# Autodesk Inventor assembly: DriverStation-ver3-1111-2021
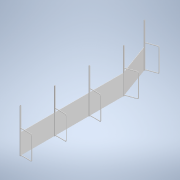
[picture p0: Inventor's stored thumbnail of the model, 180x180]
Saved by Autodesk Inventor 2021 (Build 250183000, 183)
## iProperties
Created: 2021-03-02
Part Number: DriverStation-ver3-1111-2021
Document SubType Name: Assembly
Designer: CMurray
Author: CMurray
## Documents named in this file (3)
- F:\PHRC CADD 2021\2021 Game Design Challenge\Player Station\Assemblies\DriverStation-ver3-1111-2021.iam
- F:\PHRC CADD 2021\2021 Game Design Challenge\Player Station\Parts\StationBase-ver1-1111-2021.ipt
- F:\PHRC CADD 2021\2021 Game Design Challenge\Player Station\Parts\StationDivider-ver1-1111-2021.iam
## Components (9 placed, 2 different names)
1. StationBase-ver1-1111-2021:1 — Mate:1, Flush:1, Flush:2, Flush:3, Mate:2, Flush:4, Flush:7, Flush:8, Flush:11, Flush:12
2. StationDivider-ver1-1111-2021:1 [sub-assembly] — Mate:1, Flush:1, Flush:2, Mate:6
3. StationDivider-ver1-1111-2021:2 [sub-assembly] — Flush:3, Mate:2, Flush:4, Mate:4
4. StationBase-ver1-1111-2021:2 — Mate:4, Flush:7, Flush:8, Flush:13, Mate:9, Flush:16, Angle:1
5. StationBase-ver1-1111-2021:3 — Flush:11, Flush:12, Mate:6
6. StationDivider-ver1-1111-2021:4 [sub-assembly]
7. StationBase-ver1-1111-2021:4 — Flush:13, Mate:8, Flush:14, Flush:15, Mate:10, Angle:1
8. StationDivider-ver1-1111-2021:5 [sub-assembly] — Mate:8, Flush:14, Flush:15, Angle:2
9. StationDivider-ver1-1111-2021:6 [sub-assembly] — Mate:9, Flush:16, Mate:10, Angle:2
## Relationships (24: Flush 14, Mate 8, Angle 2)
- Mate:1: StationBase-ver1-1111-2021:1 ↔ StationDivider-ver1-1111-2021:1
- Flush:1: StationBase-ver1-1111-2021:1 ↔ StationDivider-ver1-1111-2021:1
- Flush:2: StationBase-ver1-1111-2021:1 ↔ StationDivider-ver1-1111-2021:1
- Flush:3: StationBase-ver1-1111-2021:1 ↔ StationDivider-ver1-1111-2021:2
- Mate:2: StationBase-ver1-1111-2021:1 ↔ StationDivider-ver1-1111-2021:2
- Flush:4: StationBase-ver1-1111-2021:1 ↔ StationDivider-ver1-1111-2021:2
- Mate:4: StationDivider-ver1-1111-2021:2 ↔ StationBase-ver1-1111-2021:2
- Flush:7: StationBase-ver1-1111-2021:1 ↔ StationBase-ver1-1111-2021:2
- Flush:8: StationBase-ver1-1111-2021:1 ↔ StationBase-ver1-1111-2021:2
- [Mate]: StationBase-ver1-1111-2021:3 ↔ StationDivider-ver1-1111-2021:4
- [Flush]: StationBase-ver1-1111-2021:3 ↔ StationDivider-ver1-1111-2021:4
- [Flush]: StationBase-ver1-1111-2021:3 ↔ StationDivider-ver1-1111-2021:4
- Flush:11: StationBase-ver1-1111-2021:1 ↔ StationBase-ver1-1111-2021:3
- Flush:12: StationBase-ver1-1111-2021:1 ↔ StationBase-ver1-1111-2021:3
- Mate:6: StationDivider-ver1-1111-2021:1 ↔ StationBase-ver1-1111-2021:3
- Flush:13: StationBase-ver1-1111-2021:2 ↔ StationBase-ver1-1111-2021:4
- Mate:8: StationBase-ver1-1111-2021:4 ↔ StationDivider-ver1-1111-2021:5
- Flush:14: StationBase-ver1-1111-2021:4 ↔ StationDivider-ver1-1111-2021:5
- Flush:15: StationBase-ver1-1111-2021:4 ↔ StationDivider-ver1-1111-2021:5
- Mate:9: StationBase-ver1-1111-2021:2 ↔ StationDivider-ver1-1111-2021:6
- Flush:16: StationBase-ver1-1111-2021:2 ↔ StationDivider-ver1-1111-2021:6
- Mate:10: StationBase-ver1-1111-2021:4 ↔ StationDivider-ver1-1111-2021:6
- Angle:1 (20 deg): StationBase-ver1-1111-2021:2 ↔ StationBase-ver1-1111-2021:4
- Angle:2 (0 deg): StationDivider-ver1-1111-2021:5 ↔ StationDivider-ver1-1111-2021:6
## Named parameters: d12_d0 = 0 mm, d13_d1 = 0 mm, d14_d2 = 0 mm
